# Autodesk Inventor assembly: Сборка1
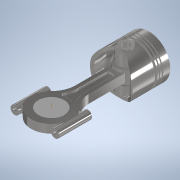
[picture p0: Inventor's stored thumbnail of the model, 180x180]
Saved by Autodesk Inventor 2021 (Build 250183000, 183)
## iProperties
Created: 2021-06-05
Part Number: Сборка1
Document SubType Name: Assembly
Designer: panda
Author: panda
## Documents named in this file (5)
- C:\Users\panda\Desktop\engine-design-hw\расчет шатуна и пальца\Сборка1.iam
- C:\Users\panda\Desktop\engine-design-hw\расчет шатуна и пальца\connecting_rod.ipt
- C:\Users\panda\Desktop\engine-design-hw\расчет шатуна и пальца\pin.ipt
- C:\Users\panda\Desktop\engine-design-hw\расчет шатуна и пальца\Бублик.ipt
- C:\Users\panda\Desktop\engine-design-hw\расчет шатуна и пальца\piston.ipt
## Components (4 placed, 4 different names)
1. connecting_rod:1 — Совмещение:1, Совмещение:2, Совмещение:3, Угол:1
2. pin:1 — Совмещение:1, Совмещение:2, Совмещение:4
3. Бублик:1 — Совмещение:3
4. piston:1 — Угол:1, Совмещение:4
## Relationships (5: Mate 4, Angle 1)
- Совмещение:1 [Mate]: connecting_rod:1 ↔ pin:1
- Совмещение:2 [Mate] (31.5 mm): connecting_rod:1 ↔ pin:1
- Совмещение:3 [Mate]: connecting_rod:1 ↔ Бублик:1
- Угол:1 [Angle] (0 deg): connecting_rod:1 ↔ piston:1
- Совмещение:4 [Mate]: pin:1 ↔ piston:1
